# Autodesk Inventor assembly: 6-HiGrip-am-0940
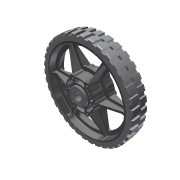
[picture p0: Inventor's stored thumbnail of the model, 180x180]
Saved by Autodesk Inventor 2012 (Build 160160000, 160)
## iProperties
Created: 2012-01-08
Part Number: 6-HiGrip-am-0940
Document SubType Name: Assembly
Designer: JesseK
Mass: 305.945 g
Surface Area: 1170.57 cm^2
Volume: 198.253 cm^3
Density: 1.5432 g/cm^3
Translation Standard: STEP AP203
FileName: 6-HiGrip-am-0940.STEP
PreProcessor: SolidWorks 2010
PostProcessor: Build: 160, Release: 2012 RTM - Date: Tue 03/01/2011
Sent Units: inch
Uncertainty: 1e-05
Author: JesseK
## Documents named in this file (4)
- Z:\UserData\Documents\Inventor\team1885frc\AndyMark\HiGrip6in\6-HiGrip-am-0940.iam
- Z:\UserData\Documents\Inventor\team1885frc\AndyMark\HiGrip6in\Imported Components\6-HiGrip-am-0940\6in 2008 FIRST Hub.ipt
- Z:\UserData\Documents\Inventor\team1885frc\AndyMark\HiGrip6in\Imported Components\6-HiGrip-am-0940\6 HiGrip Tread.ipt
- Z:\UserData\Documents\Inventor\team1885frc\Hardware\Bearings\Bearing_0.375ID_1.125OD.ipt
## Components (4 placed, 3 different names)
1. 6in 2008 FIRST Hub:1 — Mate:1, Mate:2, Mate:3, Mate:4
2. 6 HiGrip Tread:1
3. Bearing_0.375ID_1.125OD:1 — Mate:3, Mate:4
4. Bearing_0.375ID_1.125OD:2 — Mate:1, Mate:2
## Relationships (4: Mate 4)
- Mate:1: 6in 2008 FIRST Hub:1 ↔ Bearing_0.375ID_1.125OD:2
- Mate:2: 6in 2008 FIRST Hub:1 ↔ Bearing_0.375ID_1.125OD:2
- Mate:3: 6in 2008 FIRST Hub:1 ↔ Bearing_0.375ID_1.125OD:1
- Mate:4: 6in 2008 FIRST Hub:1 ↔ Bearing_0.375ID_1.125OD:1
